# Autodesk Inventor assembly: Sideways pulley mount 2
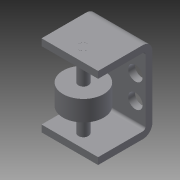
[picture p0: Inventor's stored thumbnail of the model, 180x180]
Saved by Autodesk Inventor 2013 (Build 170138000, 138)
## iProperties
Created: 2013-02-07
Part Number: Sideways pulley mount 2
Document SubType Name: Assembly
Designer: Arpan
Author: Arpan
## Documents named in this file (4)
- C:\Users\Moses\Documents\GitHub\frc2013CAD\Cimber actual\Sideways pulley mount 2.iam
- C:\Users\Moses\Documents\GitHub\frc2013CAD\Cimber actual\3 16ths shaft.ipt
- C:\Users\Moses\Documents\GitHub\frc2013CAD\Cimber actual\1 8th pulley.ipt
- C:\Users\Moses\Documents\GitHub\frc2013CAD\Cimber actual\pulley mount actual sideways left.ipt
## Components (3 placed, 3 different names)
1. 3 16ths shaft:1 — Mate:2, Mate:3, Flush:1
2. 1 8th pulley:1 — Mate:2, Mate:4
3. pulley mount actual sideways left:1 — Mate:3, Flush:1, Mate:4
## Relationships (4: Mate 3, Flush 1)
- Mate:2: 3 16ths shaft:1 ↔ 1 8th pulley:1
- Mate:3: 3 16ths shaft:1 ↔ pulley mount actual sideways left:1
- Flush:1: 3 16ths shaft:1 ↔ pulley mount actual sideways left:1
- Mate:4 (11.2268 mm): 1 8th pulley:1 ↔ pulley mount actual sideways left:1
